# Autodesk Inventor assembly: Baugruppe1
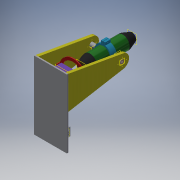
[picture p0: Inventor's stored thumbnail of the model, 180x180]
Saved by Autodesk Inventor 2017 (Build 210142000, 142)
## iProperties
Part Number: Baugruppe1
Material: Generisch
Document SubType Name: Assembly
Designer: Fabio
Author: Fabio
## Documents named in this file (10)
- C:\Users\Fabio\dicer\inventor\Baugruppe1.iam
- C:\Users\Fabio\dicer\inventor\cylinder.ipt
- C:\Users\Fabio\dicer\inventor\endkappen.ipt
- C:\Users\Fabio\dicer\inventor\spannringe.ipt
- C:\Users\Fabio\dicer\inventor\spannring_achse.ipt
- C:\Users\Fabio\dicer\inventor\halter_seite.ipt
- C:\Users\Fabio\dicer\inventor\grundplatte.ipt
- C:\Users\Fabio\dicer\inventor\LED_Ring.ipt
- C:\Users\Fabio\dicer\inventor\spiegelhalter.ipt
- C:\Users\Fabio\dicer\inventor\kamera_dummy.ipt
## Components (13 placed, 9 different names)
1. cylinder:1 — Passend:1, Passend:2, Passend:3
2. endkappen:1 — Passend:1
3. endkappen:2 — Passend:2
4. spannringe:1 — Passend:4, Passend:5
5. spannringe:2 — Passend:3, Passend:4, Passend:6
6. spannring_achse:1 — Passend:5, Einfügen:2
7. spannring_achse:2 — Passend:6, Einfügen:1
8. halter_seite:1 — Einfügen:2, Passend:8
9. halter_seite:2 — Einfügen:1, Passend:7
10. grundplatte:1 — Passend:7, Passend:9
11. LED_Ring:1 — Passend:8
12. spiegelhalter:2 — Passend:9
13. kamera_dummy:1
## Relationships (11: Mate 9, Insert 2)
- Passend:1 [Mate]: cylinder:1 ↔ endkappen:1
- Passend:2 [Mate]: cylinder:1 ↔ endkappen:2
- Passend:3 [Mate]: cylinder:1 ↔ spannringe:2
- Passend:4 [Mate] (1 mm): spannringe:1 ↔ spannringe:2
- Passend:5 [Mate]: spannringe:1 ↔ spannring_achse:1
- Passend:6 [Mate]: spannringe:2 ↔ spannring_achse:2
- Einfügen:1 [Insert] (-10 mm): spannring_achse:2 ↔ halter_seite:2
- Einfügen:2 [Insert] (-10 mm): spannring_achse:1 ↔ halter_seite:1
- Passend:7 [Mate]: halter_seite:2 ↔ grundplatte:1
- Passend:8 [Mate]: halter_seite:1 ↔ LED_Ring:1
- Passend:9 [Mate]: grundplatte:1 ↔ spiegelhalter:2
